# Autodesk Inventor assembly: PCBPT_V3
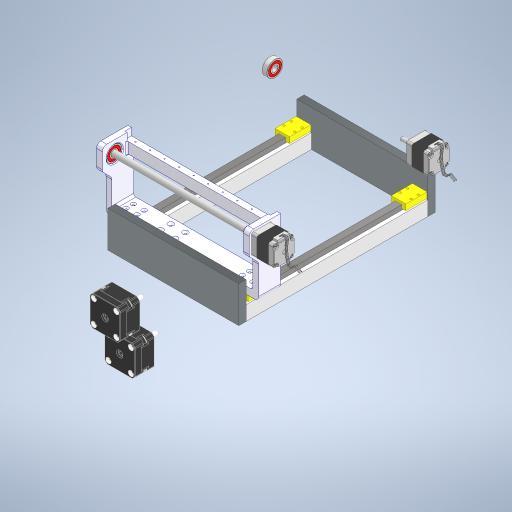
[picture p0: Inventor's stored thumbnail of the model, 512x512]
Saved by Autodesk Inventor 2024 (Build 280153000, 153)
## iProperties
Created: 2023-08-11
Part Number: PCBPT_V3
Document SubType Name: Assembly
Designer: l1534
Author: l1534
## Documents named in this file (10)
- C:\DATA\Documents\Lab\github\PCBPT\PCBPT_V3\Mechanical\PCBPT_V3.iam
- C:\DATA\Documents\Lab\github\PCBPT\PCBPT_V3\Mechanical\wall.ipt
- C:\DATA\Documents\Lab\github\PCBPT\PCBPT_V3\Mechanical\NEMA11\NEMA11.iam
- C:\DATA\Documents\Lab\github\PCBPT\PCBPT_V3\Mechanical\2020x260mm.ipt
- C:\DATA\Documents\Lab\github\PCBPT\PCBPT_V3\Mechanical\MGN9_rail.ipt
- C:\DATA\Documents\Lab\github\PCBPT\PCBPT_V3\Mechanical\MGN9C_block.ipt
- C:\DATA\Documents\Lab\github\PCBPT\PCBPT_V3\Mechanical\gantry_R.ipt
- C:\DATA\Documents\Lab\github\PCBPT\PCBPT_V3\Mechanical\608-2RS Skate Board Ball Bearing\608-2RS Skate Board Ball Bearing.iam
- C:\DATA\Documents\Lab\github\FlexiNet\mechanical\T8_Lead_screw.ipt
- C:\DATA\Documents\Lab\github\PCBPT\PCBPT_V3\Mechanical\NEMA_17_PHB42S28-406A v2\NEMA_17_PHB42S28-406A v2.ipt
## Components (18 placed, 9 different names)
1. wall:1 — Rigid:1, Rigid:2
2. 2020x250mm:1 — Rigid:1, Rigid:5
3. 2020x250mm:2 — Rigid:2, Rigid:3, Rigid:4
4. wall:2 — Rigid:3
5. MGN9_rail:1 — Rigid:4, Slider:2, Slider:3
6. MGN9_rail:2 — Rigid:5, Slider:1, Slider:4
7. MGN9C_block:1 — Slider:4, Flush:2
8. MGN9C_block:2 — Slider:2, Flush:1
9. MGN9C_block:3 — Slider:1, Flush:1, Rigid:8
10. MGN9C_block:4 — Slider:3, Flush:2
11. NEMA11:3 [sub-assembly]
12. NEMA11:4 [sub-assembly] — Insert:1, Rotational:2
13. gantry_R:1 — Rigid:8, Insert:1, Rotational:1
14. 608-2RS Skate Board Ball Bearing:1 [sub-assembly] — Rotational:1
15. 608-2RS Skate Board Ball Bearing:2 [sub-assembly]
16. T8_Lead_screw:1 — Rotational:2
17. NEMA_17_PHB42S28-406A v2:1
18. NEMA_17_PHB42S28-406A v2:2
## Relationships (15: WeldJoint 6, TranslationJoint 4, Flush 2, RevoluteJoint 2, Insert 1)
- Rigid:1 [WeldJoint]: wall:1 ↔ 2020x250mm:1
- Rigid:2 [WeldJoint]: wall:1 ↔ 2020x250mm:2
- Rigid:3 [WeldJoint]: 2020x250mm:2 ↔ wall:2
- Rigid:4 [WeldJoint]: 2020x250mm:2 ↔ MGN9_rail:1
- Rigid:5 [WeldJoint]: 2020x250mm:1 ↔ MGN9_rail:2
- Slider:1 [TranslationJoint]: MGN9_rail:2 ↔ MGN9C_block:3
- Slider:2 [TranslationJoint]: MGN9_rail:1 ↔ MGN9C_block:2
- Slider:3 [TranslationJoint]: MGN9_rail:1 ↔ MGN9C_block:4
- Slider:4 [TranslationJoint]: MGN9_rail:2 ↔ MGN9C_block:1
- Flush:1: MGN9C_block:2 ↔ MGN9C_block:3
- Flush:2: MGN9C_block:1 ↔ MGN9C_block:4
- Rigid:8 [WeldJoint]: MGN9C_block:3 ↔ gantry_R:1
- Insert:1: NEMA11:4 ↔ gantry_R:1
- Rotational:1 [RevoluteJoint]: gantry_R:1 ↔ 608-2RS Skate Board Ball Bearing:1
- Rotational:2 [RevoluteJoint]: NEMA11:4 ↔ T8_Lead_screw:1
